# Autodesk Inventor assembly: 203.003.01_ZB_Geranulatvorfuehrung
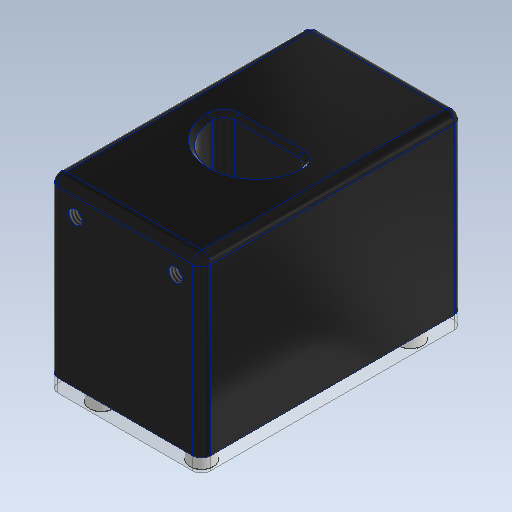
[picture p0: Inventor's stored thumbnail of the model, 512x512]
Saved by Autodesk Inventor 2021 (Build 250183000, 183)
## iProperties
Created: 2021-10-30
Part Number: 203.003.01_ZB_Geranulatvorfuehrung
Document SubType Name: Assembly
Designer: Sebastian Seewald
Author: Sebastian Seewald
## Documents named in this file (4)
- C:\Users\Sebastian Seewald\Documents\Inventor\Konstruktion_Studium\Lernfabrik\104_Extrudereinheit\204.004.01_ZB_Geranulatvorfuehrung.iam
- C:\Users\Sebastian Seewald\Documents\Inventor\Konstruktion_Studium\Lernfabrik\104_Extrudereinheit\104.002.01_Gehaeuse_Granulatfuehrung.ipt
- C:\Users\Sebastian Seewald\Documents\Inventor\Konstruktion_Studium\Lernfabrik\104_Extrudereinheit\104.011.01_Abdeckplatte_Extruderfuehrung.ipt
- C:\Users\Sebastian Seewald\Documents\Inventor\Konstruktion_Studium\Lernfabrik\104_Extrudereinheit\Schrauben\DIN 912 - M3 x 8.ipt
## Components (6 placed, 3 different names)
1. 104.002.01_Gehaeuse_Granulatfuehrung:1 — Passend:1, Fluchtend:1, Fluchtend:2
2. 104.011.01_Abdeckplatte_Extruderfuehrung:1 — Passend:1, Fluchtend:1, Fluchtend:2, Passend:2, Passend:3, Passend:4, Passend:5, Passend:6, Passend:7, Passend:8, Passend:9
3. DIN 912 - M3 x 8:1 — Passend:2, Passend:6
4. DIN 912 - M3 x 8:2 — Passend:3, Passend:8
5. DIN 912 - M3 x 8:3 — Passend:4, Passend:9
6. DIN 912 - M3 x 8:4 — Passend:5, Passend:7
## Relationships (11: Mate 9, Flush 2)
- Passend:1 [Mate]: 104.002.01_Gehaeuse_Granulatfuehrung:1 ↔ 104.011.01_Abdeckplatte_Extruderfuehrung:1
- Fluchtend:1 [Flush]: 104.002.01_Gehaeuse_Granulatfuehrung:1 ↔ 104.011.01_Abdeckplatte_Extruderfuehrung:1
- Fluchtend:2 [Flush]: 104.002.01_Gehaeuse_Granulatfuehrung:1 ↔ 104.011.01_Abdeckplatte_Extruderfuehrung:1
- Passend:2 [Mate]: 104.011.01_Abdeckplatte_Extruderfuehrung:1 ↔ DIN 912 - M3 x 8:1
- Passend:3 [Mate]: 104.011.01_Abdeckplatte_Extruderfuehrung:1 ↔ DIN 912 - M3 x 8:2
- Passend:4 [Mate]: 104.011.01_Abdeckplatte_Extruderfuehrung:1 ↔ DIN 912 - M3 x 8:3
- Passend:5 [Mate]: 104.011.01_Abdeckplatte_Extruderfuehrung:1 ↔ DIN 912 - M3 x 8:4
- Passend:6 [Mate]: 104.011.01_Abdeckplatte_Extruderfuehrung:1 ↔ DIN 912 - M3 x 8:1
- Passend:7 [Mate]: 104.011.01_Abdeckplatte_Extruderfuehrung:1 ↔ DIN 912 - M3 x 8:4
- Passend:8 [Mate]: 104.011.01_Abdeckplatte_Extruderfuehrung:1 ↔ DIN 912 - M3 x 8:2
- Passend:9 [Mate]: 104.011.01_Abdeckplatte_Extruderfuehrung:1 ↔ DIN 912 - M3 x 8:3
